# Autodesk Inventor assembly: Screw Assembly
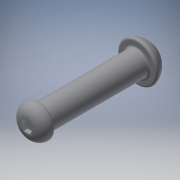
[picture p0: Inventor's stored thumbnail of the model, 180x180]
Saved by Autodesk Inventor 2018 (Build 220112000, 112)
## iProperties
Created: 2018-04-09
Part Number: Screw Assembly
Document SubType Name: Assembly
Designer: 232963
Author: 232963
## Documents named in this file (3)
- P:\IED\SchoolCAD\Design Challenge\Screw Assembly.iam
- P:\IED\SchoolCAD\Design Challenge\Screw.ipt
- P:\IED\SchoolCAD\Design Challenge\Part3.ipt
## Components (2 placed, 2 different names)
1. Screw:1 — Insert:1
2. Part3:1 — Insert:1
## Relationships (1: Insert 1)
- Insert:1: Screw:1 ↔ Part3:1
